# Autodesk Inventor assembly: StereoPiM12
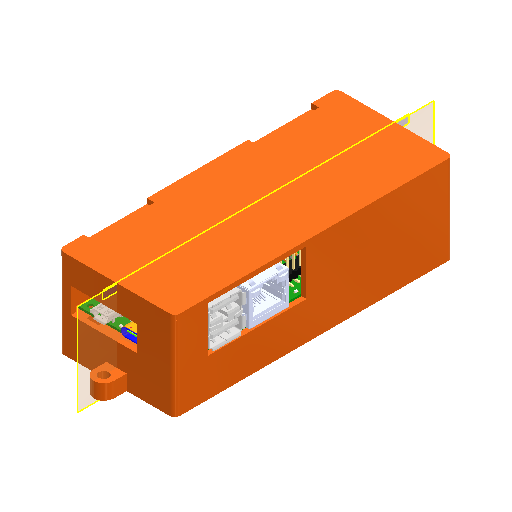
[picture p0: Inventor's stored thumbnail of the model, 512x512]
Saved by Autodesk Inventor 2025.2 (Build 292293000, 293)
## iProperties
Created: 2026-05-15
Part Number: StereoPiM12
Document SubType Name: Assembly
Designer: rolan
Author: rolan
## Documents named in this file (4)
- C:\Users\rolan\Documents\PhD\Inventor\Assembly\StereoPiM12.iam
- C:\Users\rolan\Documents\PhD\Inventor\Parts\M12StereoPiBracket.ipt
- C:\Users\rolan\Documents\PhD\Inventor\3D Files\stereopi_v2\stereopi_v2\stereopi_v2.ipt
- C:\Users\rolan\Documents\PhD\Inventor\Parts\StereoPiBracketLidM12.ipt
## Components (3 placed, 3 different names)
1. M12StereoPiBracket:1 — Mate:1, Mate:2, Mate:3, Mate:4, Mate:5, Mate:6
2. stereopi_v2:1 — Mate:1, Mate:2, Mate:3
3. StereoPiBracketLidM12:1 — Mate:4, Mate:5, Mate:6
## Relationships (6: Mate 6)
- Mate:1: M12StereoPiBracket:1 ↔ stereopi_v2:1
- Mate:2: M12StereoPiBracket:1 ↔ stereopi_v2:1
- Mate:3: M12StereoPiBracket:1 ↔ stereopi_v2:1
- Mate:4: M12StereoPiBracket:1 ↔ StereoPiBracketLidM12:1
- Mate:5: M12StereoPiBracket:1 ↔ StereoPiBracketLidM12:1
- Mate:6: M12StereoPiBracket:1 ↔ StereoPiBracketLidM12:1
